# Autodesk Inventor assembly: SubSistemaLiberacion
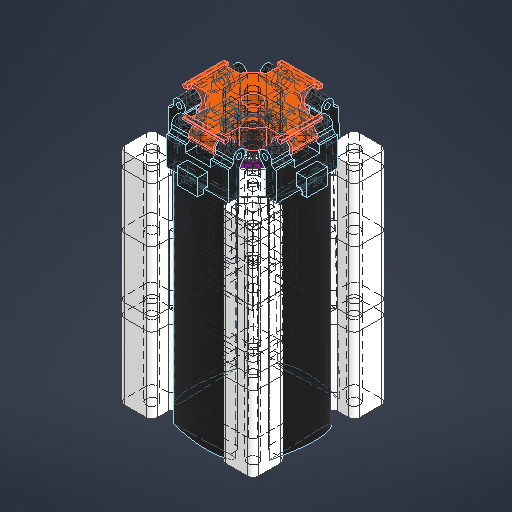
[picture p0: Inventor's stored thumbnail of the model, 512x512]
Saved by Autodesk Inventor 2026.1 (Build 301233000, 233)
## iProperties
Created: 2025-12-08
Part Number: SubSistemaLiberacion
Document SubType Name: Assembly
Designer: vickh
Author: vickh
## Documents named in this file (12)
- C:\Users\vickh\Documents\Proyectos\Cansat_Huitzilin\3D\NuevoDiseno\SubSistemaLiberacion.iam
- C:\Users\vickh\Documents\Proyectos\Cansat_Huitzilin\3D\NuevoDiseno\SujeccionHelices.ipt
- C:\Users\vickh\Documents\Proyectos\Cansat_Huitzilin\3D\NuevoDiseno\expansor de conexion.ipt
- C:\Users\vickh\Downloads\Bearing 625 2RS\Bearing 625 2RS\Bearing 625 2RS.ipt
- C:\Users\vickh\Documents\Proyectos\Cansat_Huitzilin\3D\NuevoDiseno\Pala.ipt
- C:\Users\vickh\Documents\Proyectos\Cansat_Huitzilin\3D\NuevoDiseno\SistemaLiberacion2.2.ipt
- C:\Users\vickh\Documents\Proyectos\Cansat_Huitzilin\3D\NuevoDiseno\SistemLiberacion1.ipt
- C:\Users\vickh\Documents\Proyectos\Cansat_Huitzilin\3D\NuevoDiseno\InsertoM3.ipt
- C:\Users\vickh\Documents\Proyectos\Cansat_Huitzilin\3D\NuevoDiseno\Electronica.ipt
- C:\Users\vickh\Documents\Proyectos\Cansat_Huitzilin\3D\NuevoDiseno\SemillasyAgua.ipt
- C:\Users\vickh\Documents\Proyectos\Cansat_Huitzilin\3D\NuevoDiseno\Huevo.ipt
- C:\Users\vickh\Documents\Proyectos\Cansat_Huitzilin\3D\NuevoDiseno\TornilloM3.ipt
## Components (16 placed, 11 different names)
1. SujeccionHelices:1 — Insertar:1, De rotación:1, De rotación:2, De rotación:3, De rotación:4
2. expansor de conexion:1 — Insertar:2, Insertar:3, Coincidencia:1, Insertar:4
3. Bearing 625 2RS:1 — Insertar:1, Insertar:2
4. Pala:1 — De rotación:1
5. Pala:2 — De rotación:3
6. Pala:3 — De rotación:4
7. Pala:4 — De rotación:2
8. SistemaLiberacion2.2:1 — Insertar:3, Cilíndrica:1, Coincidencia:2, Nivelación:1, Nivelación:2
9. SistemLiberacion1:1 — Cilíndrica:1
10. InsertoM3:1 — Coincidencia:1, Cilíndrica:2
11. InsertoM3:2 — Insertar:4, Cilíndrica:3
12. Electronica:1 — Coincidencia:2, Nivelación:1, Nivelación:2, Coincidencia:3, Nivelación:3, Nivelación:4
13. SemillasyAgua:1 — Coincidencia:3, Nivelación:3, Nivelación:4, Coincidencia:4, Nivelación:5, Nivelación:6
14. Huevo:1 — Coincidencia:4, Nivelación:5, Nivelación:6
15. TornilloM3:1 — Cilíndrica:2
16. TornilloM3:2 — Cilíndrica:3
## Relationships (21: Flush 6, Insert 4, RevoluteJoint 4, Mate 4, CylindricalJoint 3)
- Insertar:1: SujeccionHelices:1 ↔ Bearing 625 2RS:1
- Insertar:2: expansor de conexion:1 ↔ Bearing 625 2RS:1
- De rotación:1 [RevoluteJoint]: SujeccionHelices:1 ↔ Pala:1
- De rotación:2 [RevoluteJoint]: SujeccionHelices:1 ↔ Pala:4
- De rotación:3 [RevoluteJoint]: SujeccionHelices:1 ↔ Pala:2
- De rotación:4 [RevoluteJoint]: SujeccionHelices:1 ↔ Pala:3
- Insertar:3 (0.1 mm): expansor de conexion:1 ↔ SistemaLiberacion2.2:1
- Cilíndrica:1 [CylindricalJoint]: SistemaLiberacion2.2:1 ↔ SistemLiberacion1:1
- Coincidencia:1 [Mate]: expansor de conexion:1 ↔ InsertoM3:1
- Insertar:4: expansor de conexion:1 ↔ InsertoM3:2
- Coincidencia:2 [Mate]: SistemaLiberacion2.2:1 ↔ Electronica:1
- Nivelación:1 [Flush]: SistemaLiberacion2.2:1 ↔ Electronica:1
- Nivelación:2 [Flush]: SistemaLiberacion2.2:1 ↔ Electronica:1
- Coincidencia:3 [Mate]: Electronica:1 ↔ SemillasyAgua:1
- Nivelación:3 [Flush]: Electronica:1 ↔ SemillasyAgua:1
- Nivelación:4 [Flush]: Electronica:1 ↔ SemillasyAgua:1
- Coincidencia:4 [Mate]: SemillasyAgua:1 ↔ Huevo:1
- Nivelación:5 [Flush]: SemillasyAgua:1 ↔ Huevo:1
- Nivelación:6 [Flush]: SemillasyAgua:1 ↔ Huevo:1
- Cilíndrica:2 [CylindricalJoint]: InsertoM3:1 ↔ TornilloM3:1
- Cilíndrica:3 [CylindricalJoint]: InsertoM3:2 ↔ TornilloM3:2
